# Autodesk Inventor assembly: ASTRAIOSAssembly
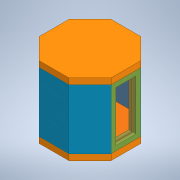
[picture p0: Inventor's stored thumbnail of the model, 180x180]
Saved by Autodesk Inventor 2020 (Build 240168000, 168)
## iProperties
Created: 2020-02-24
Part Number: ASTRAIOSAssembly
Document SubType Name: Assembly
Designer: WANG
Author: WANG
## Documents named in this file (6)
- C:\Users\ianwa\Documents\GitHub\ASTRAIOS\workspace\ASTRAIOSAssembly.iam
- C:\Users\ianwa\Documents\GitHub\ASTRAIOS\workspace\SatelliteTopFace.ipt
- C:\Users\ianwa\Documents\GitHub\ASTRAIOS\workspace\SatelliteBottomFace.ipt
- C:\Users\ianwa\Documents\GitHub\ASTRAIOS\workspace\SatelliteSideWallSensor.ipt
- C:\Users\ianwa\Documents\GitHub\ASTRAIOS\workspace\SatelliteSideWallFilled.ipt
- C:\Users\ianwa\Documents\GitHub\ASTRAIOS\workspace\SatelliteLexanPlateSensor.ipt
## Components (11 placed, 5 different names)
1. SatelliteBottomFace:1 — Flush:1, Flush:2, Flush:3, Flush:4, Mate:1, Mate:3, Mate:5, Mate:8, Mate:11, Mate:15, Mate:18, Mate:19, Mate:20, Mate:23
2. SatelliteTopFace:2 — Flush:1, Flush:2, Flush:3, Flush:4, Mate:1, Mate:2, Mate:4, Mate:6, Mate:10, Mate:13, Mate:16, Mate:22, Mate:25
3. SatelliteSideWallSensor:1 — Mate:2, Mate:3, Mate:4, Mate:7, Mate:9, Mate:26, Mate:27, Mate:28
4. SatelliteSideWallFilled:1 — Mate:8, Mate:9, Mate:10, Mate:12
5. SatelliteSideWallFilled:2 — Mate:11, Mate:12, Mate:13, Mate:14
6. SatelliteSideWallFilled:3 — Mate:5, Mate:6, Mate:7, Mate:24
7. SatelliteSideWallFilled:4 — Mate:17, Mate:18, Mate:19, Mate:21
8. SatelliteSideWallFilled:5 — Mate:14, Mate:15, Mate:16, Mate:17
9. SatelliteSideWallFilled:6 — Mate:20, Mate:21, Mate:22
10. SatelliteSideWallFilled:7 — Mate:23, Mate:24, Mate:25
11. SatelliteLexanPlateSensor:1 — Mate:26, Mate:27, Mate:28
## Relationships (32: Mate 28, Flush 4)
- Flush:1: SatelliteBottomFace:1 ↔ SatelliteTopFace:2
- Flush:2: SatelliteBottomFace:1 ↔ SatelliteTopFace:2
- Flush:3: SatelliteBottomFace:1 ↔ SatelliteTopFace:2
- Flush:4: SatelliteBottomFace:1 ↔ SatelliteTopFace:2
- Mate:1 (114.3 mm): SatelliteBottomFace:1 ↔ SatelliteTopFace:2
- Mate:2: SatelliteTopFace:2 ↔ SatelliteSideWallSensor:1
- Mate:3: SatelliteBottomFace:1 ↔ SatelliteSideWallSensor:1
- Mate:4: SatelliteTopFace:2 ↔ SatelliteSideWallSensor:1
- Mate:5: SatelliteBottomFace:1 ↔ SatelliteSideWallFilled:3
- Mate:6: SatelliteTopFace:2 ↔ SatelliteSideWallFilled:3
- Mate:7: SatelliteSideWallSensor:1 ↔ SatelliteSideWallFilled:3
- Mate:8: SatelliteBottomFace:1 ↔ SatelliteSideWallFilled:1
- Mate:9: SatelliteSideWallSensor:1 ↔ SatelliteSideWallFilled:1
- Mate:10: SatelliteTopFace:2 ↔ SatelliteSideWallFilled:1
- Mate:11: SatelliteBottomFace:1 ↔ SatelliteSideWallFilled:2
- Mate:12: SatelliteSideWallFilled:1 ↔ SatelliteSideWallFilled:2
- Mate:13: SatelliteTopFace:2 ↔ SatelliteSideWallFilled:2
- Mate:14: SatelliteSideWallFilled:2 ↔ SatelliteSideWallFilled:5
- Mate:15: SatelliteBottomFace:1 ↔ SatelliteSideWallFilled:5
- Mate:16: SatelliteTopFace:2 ↔ SatelliteSideWallFilled:5
- Mate:17: SatelliteSideWallFilled:4 ↔ SatelliteSideWallFilled:5
- Mate:18: SatelliteBottomFace:1 ↔ SatelliteSideWallFilled:4
- Mate:19: SatelliteBottomFace:1 ↔ SatelliteSideWallFilled:4
- Mate:20: SatelliteBottomFace:1 ↔ SatelliteSideWallFilled:6
- Mate:21: SatelliteSideWallFilled:4 ↔ SatelliteSideWallFilled:6
- Mate:22: SatelliteTopFace:2 ↔ SatelliteSideWallFilled:6
- Mate:23: SatelliteBottomFace:1 ↔ SatelliteSideWallFilled:7
- Mate:24: SatelliteSideWallFilled:3 ↔ SatelliteSideWallFilled:7
- Mate:25: SatelliteTopFace:2 ↔ SatelliteSideWallFilled:7
- Mate:26: SatelliteSideWallSensor:1 ↔ SatelliteLexanPlateSensor:1
- Mate:27: SatelliteSideWallSensor:1 ↔ SatelliteLexanPlateSensor:1
- Mate:28: SatelliteSideWallSensor:1 ↔ SatelliteLexanPlateSensor:1
